# Autodesk Inventor assembly: Bumpers
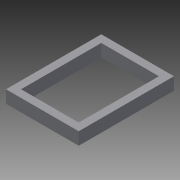
[picture p0: Inventor's stored thumbnail of the model, 180x180]
Saved by Autodesk Inventor 2013 (Build 170138000, 138)
## iProperties
Created: 2014-01-18
Part Number: Bumpers
Document SubType Name: Assembly
Designer: 215152
Author: 215152
## Documents named in this file (3)
- F:\Robotics\FRC\2014\CAD\Robot\Bumpers\Bumpers.iam
- F:\Robotics\FRC\2014\CAD\Brian's Derp\Additions\BumperFront.ipt
- F:\Robotics\FRC\2014\CAD\Brian's Derp\Additions\BumperSide.ipt
## Components (4 placed, 2 different names)
1. BumperFront:1 — Mate:1, Mate:2, Flush:1, Flush:2, Flush:3, Flush:4, Flush:5
2. BumperFront:2 — Flush:5, Mate:3, Flush:6
3. BumperSide:1 — Mate:1, Flush:2, Flush:4, Mate:3, Flush:6
4. BumperSide:2 — Mate:2, Flush:1, Flush:3
## Relationships (9: Flush 6, Mate 3)
- Mate:1: BumperFront:1 ↔ BumperSide:1
- Mate:2: BumperFront:1 ↔ BumperSide:2
- Flush:1: BumperFront:1 ↔ BumperSide:2
- Flush:2: BumperFront:1 ↔ BumperSide:1
- Flush:3: BumperFront:1 ↔ BumperSide:2
- Flush:4: BumperFront:1 ↔ BumperSide:1
- Flush:5: BumperFront:1 ↔ BumperFront:2
- Mate:3: BumperFront:2 ↔ BumperSide:1
- Flush:6: BumperFront:2 ↔ BumperSide:1
